# Autodesk Inventor assembly: McCrea_head_walle
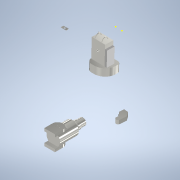
[picture p0: Inventor's stored thumbnail of the model, 180x180]
Saved by Autodesk Inventor 2022 (Build 260153000, 153)
## iProperties
Created: 2022-01-20
Part Number: McCrea_head_walle
Document SubType Name: Assembly
Designer: MatusBarany
Author: MatusBarany
## Documents named in this file (13)
- C:\Users\Max\Documents\Škola\teg\wall-e\assembly\McCrea_head_walle.iam
- C:\Users\Max\Documents\Škola\teg\wall-e\maxo\McCrea_kabel_walle.ipt
- C:\Users\Max\Documents\Škola\teg\wall-e\maxo\McCrea_krk_walle.ipt
- C:\Users\Max\Documents\Škola\teg\wall-e\maxo\McCrea_oblucik_walle.ipt
- C:\Users\Max\Documents\Škola\teg\wall-e\maxo\McCrea_oko_walle.ipt
- C:\Users\Max\Documents\Škola\teg\wall-e\maxo\McCrea_palicka_walle.ipt
- C:\Users\Max\Documents\Škola\teg\wall-e\maxo\McCrea_uhco_walle.ipt
- C:\Users\Max\Documents\Škola\teg\wall-e\maxo\McCrea_velka_palicka_walle.ipt
- C:\Users\Max\Documents\Škola\teg\wall-e\maxo\McCrea_velka_palicka_walle_1.ipt
- C:\Users\Max\Documents\Škola\teg\wall-e\maxo\McCrea_velky_krk_walle.ipt
- C:\Users\Max\Documents\Škola\teg\wall-e\maxo\McCrea_zadna_cast_oka_walle.ipt
- C:\Users\Max\Documents\Škola\teg\wall-e\maxo\McCrea_zadne_oko_walle.ipt
- C:\Users\Max\Documents\Škola\teg\wall-e\maxo\McCrea_doska_walle.ipt
## Components (15 placed, 12 different names)
1. McCrea_krk_walle:1 — Rigid:1, Rigid:2
2. McCrea_oblucik_walle:1 — Rotational:2, Rigid:2
3. McCrea_palicka_walle:1 — Rotational:1
4. McCrea_uhco_walle:1 — Mate:2, Flush:1
5. McCrea_zadna_cast_oka_walle:1 — Rigid:3, Mate:1
6. McCrea_kabel_walle:2 — Mate:3
7. McCrea_oblucik_walle:2 — Rotational:1, Rigid:1
8. McCrea_oko_walle:2 — Rigid:3
9. McCrea_palicka_walle:2 — Rotational:2
10. McCrea_velka_palicka_walle:2
11. McCrea_velka_palicka_walle_1:2 — Rotational:3
12. McCrea_velky_krk_walle:2
13. McCrea_zadne_oko_walle:2 — Mate:1, Mate:2, Flush:1, Mate:3, Rotational:3, Mate:4
14. McCrea_kabel_walle:3 — Mate:4
15. McCrea_doska_walle:1
## Relationships (11: Mate 4, RevoluteJoint 3, WeldJoint 3, Flush 1)
- Rotational:1 [RevoluteJoint]: McCrea_palicka_walle:1 ↔ McCrea_oblucik_walle:2
- Rigid:1 [WeldJoint]: McCrea_krk_walle:1 ↔ McCrea_oblucik_walle:2
- Rotational:2 [RevoluteJoint]: McCrea_oblucik_walle:1 ↔ McCrea_palicka_walle:2
- Rigid:2 [WeldJoint]: McCrea_krk_walle:1 ↔ McCrea_oblucik_walle:1
- Rigid:3 [WeldJoint]: McCrea_zadna_cast_oka_walle:1 ↔ McCrea_oko_walle:2
- Mate:1: McCrea_zadna_cast_oka_walle:1 ↔ McCrea_zadne_oko_walle:2
- Mate:2: McCrea_uhco_walle:1 ↔ McCrea_zadne_oko_walle:2
- Flush:1: McCrea_uhco_walle:1 ↔ McCrea_zadne_oko_walle:2
- Mate:3: McCrea_kabel_walle:2 ↔ McCrea_zadne_oko_walle:2
- Rotational:3 [RevoluteJoint]: McCrea_velka_palicka_walle_1:2 ↔ McCrea_zadne_oko_walle:2
- Mate:4: McCrea_zadne_oko_walle:2 ↔ McCrea_kabel_walle:3
